# Autodesk Inventor assembly: main room, doors, corridor connected
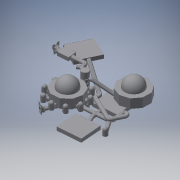
[picture p0: Inventor's stored thumbnail of the model, 180x180]
Saved by Autodesk Inventor 2017 (Build 210142000, 142)
## iProperties
Created: 2018-03-04
Part Number: main room, doors, corridor connected
Document SubType Name: Assembly
Designer: Braxton
Author: Braxton
## Documents named in this file (21)
- E:\School\Game develpment\geoscape\done solid\map (one wall)\main room, doors, corridor connected (one wall).iam
- E:\School\Game develpment\geoscape\done solid\rooms  (one wall)\assembly\main room with double door.iam
- E:\School\Game develpment\geoscape\done solid\doors\end door\9 foot door\end door room (9).ipt
- E:\School\Game develpment\geoscape\done solid\doors\end door\9 foot door\end door assembly (closed) (9).ipt.iam
- E:\School\Game develpment\geoscape\done solid\corridors (one wall done)\corridor (one wall).ipt
- E:\School\Game develpment\geoscape\done solid\corridors (one wall done)\corridor turn (one wall).ipt
- E:\School\Game develpment\geoscape\done solid\corridors (one wall done)\Y corridor  (one wall).ipt
- E:\School\Game develpment\geoscape\done solid\corridors (one wall done)\end cap (one wall).ipt
- E:\School\Game develpment\geoscape\done solid\corridors (one wall done)\curve ramp (one wall).ipt
- E:\School\Game develpment\geoscape\done solid\corridors (one wall done)\ramp top connect  (one wall).ipt
- E:\School\Game develpment\geoscape\done solid\corridors (one wall done)\ramp (one wall).ipt
- E:\School\Game develpment\geoscape\done solid\corridors (one wall done)\ramp bottom connect (one wall).ipt
- E:\School\Game develpment\geoscape\done solid\rooms  (one wall)\assembly\assembly of dome with corridors with all doors.iam
- E:\School\Game develpment\geoscape\done solid\rooms  (one wall)\assembly\dome one terminal.iam
- E:\School\Game develpment\geoscape\done solid\corridors (one wall done)\X corridor  (one wall).ipt
- E:\School\Game develpment\geoscape\done solid\corridors (one wall done)\ramp connect both ends  (one wall).ipt
- E:\School\Game develpment\geoscape\done solid\rooms  (one wall)\room with 15 cubicals (one wall).ipt
- E:\School\Game develpment\geoscape\done solid\doors\end door\9 foot door\end door assembly (9).ipt.iam
- E:\School\Game develpment\geoscape\done solid\rooms  (one wall)\assembly\dome with double door.iam
- end door assembly (closed) (9).ipt
- end door assembly (9).ipt
## Components (70 placed, 18 different names)
1. corridor (one wall):19 — Flush:52, Mate:15, Insert:66, Insert:67
2. corridor (one wall):18 — Flush:51, Flush:52, Insert:65, Insert:66
3. corridor (one wall):17 — Flush:50, Flush:51, Insert:64, Insert:65
4. corridor (one wall):16 — Flush:49, Flush:50, Insert:63, Insert:64
5. corridor (one wall):15 — Flush:48, Flush:49, Insert:62, Insert:63
6. corridor turn (one wall):8 — Mate:14, Flush:48, Insert:61, Insert:62
7. ramp top connect  (one wall):3 — Flush:47, Insert:57, Insert:60, Mate:11
8. ramp (one wall):8 — Flush:46, Flush:47, Insert:56, Insert:57
9. ramp (one wall):7 — Flush:45, Flush:46, Insert:55, Insert:56
10. ramp (one wall):6 — Flush:44, Flush:45, Insert:54, Insert:55
11. ramp (one wall):5 — Flush:43, Flush:44, Insert:53, Insert:54
12. ramp (one wall):4 — Flush:42, Flush:43, Insert:52, Insert:53
13. ramp bottom connect (one wall):3 — Insert:51, Flush:42, Insert:52
14. corridor turn (one wall):7 — Insert:49, Flush:41, Insert:51
15. corridor turn (one wall):6 — Insert:49, Insert:50, Flush:40, Flush:41
16. corridor (one wall):14 — Flush:36, Insert:48, Insert:50, Flush:40
17. corridor (one wall):13 — Flush:36, Flush:37, Insert:47, Insert:48
18. corridor (one wall):12 — Flush:37, Flush:38, Insert:46, Insert:47
19. corridor (one wall):11 — Flush:38, Flush:39, Insert:45, Insert:46
20. corridor (one wall):10 — Flush:39, Insert:44, Insert:45
21. corridor turn (one wall):5 — Flush:34, Insert:42, Insert:44
22. corridor (one wall):9 — Flush:33, Flush:34, Insert:41, Insert:42
23. corridor (one wall):8 — Flush:32, Flush:33, Insert:40, Insert:41
24. corridor turn (one wall):4 — Flush:31, Flush:32, Insert:39, Insert:40
25. corridor turn (one wall):3 — Flush:30, Flush:31, Insert:38, Insert:39
26. ramp top connect  (one wall):2 — Insert:37, Flush:29, Flush:30, Insert:38
27. ramp bottom connect (one wall):2 — Insert:37, Flush:29, Insert:43, Flush:35
28. corridor (one wall):7 — Insert:35, Flush:28, Mate:10
29. corridor (one wall):6 — Insert:34, Insert:35, Flush:27, Flush:28
30. Y corridor  (one wall):2 — Insert:33, Flush:26, Insert:34, Flush:27, Insert:43, Flush:35
31. corridor (one wall):5 — Insert:32, Insert:33, Flush:25, Flush:26
32. ramp connect both ends  (one wall):2 — Insert:30, Flush:24, Insert:58, Mate:12
33. ramp connect both ends  (one wall):1 — Insert:29, Flush:23, Insert:59, Mate:13
34. X corridor  (one wall):1 — Insert:28, Insert:29, Insert:30, Flush:22, Flush:23, Flush:24, Insert:32, Flush:25
35. corridor (one wall):4 — Insert:27, Insert:28, Flush:21, Flush:22
36. corridor (one wall):3 — Insert:26, Insert:27, Flush:20, Flush:21
37. corridor turn (one wall):2 — Insert:26, Insert:31, Mate:9, Flush:20
38. end cap (one wall):3 — Insert:25, Mate:8
39. end cap (one wall):2 — Insert:24, Mate:7
40. ramp bottom connect (one wall):1 — Insert:12, Flush:9, Insert:78, Mate:18
41. ramp (one wall):3 — Insert:11, Flush:8, Insert:12, Flush:9
42. ramp (one wall):2 — Insert:10, Insert:11, Flush:7, Flush:8
43. ramp (one wall):1 — Insert:9, Insert:10, Flush:6, Flush:7
44. ramp top connect  (one wall):1 — Insert:8, Mate:5, Insert:9, Flush:6
45. curve ramp (one wall):1 — Insert:7, Mate:4, Insert:8, Mate:5, Flush:10, Insert:24, Mate:7, Insert:25, Mate:8, Insert:31, Mate:9, Mate:14, Insert:61, Insert:77
46. end cap (one wall):1 — Insert:6, Flush:5
47. Y corridor  (one wall):1 — Insert:5, Flush:4, Insert:6, Flush:5, Insert:7, Mate:4
48. corridor turn (one wall):1 — Insert:4, Flush:3, Insert:5, Flush:4
49. corridor (one wall):2 — Insert:3, Flush:2, Insert:4, Flush:3
50. corridor (one wall):1 — Insert:2, Insert:3, Mate:3, Flush:2
51. room with 15 cubicals (one wall):1 — Insert:58, Mate:12
52. room with 15 cubicals (one wall):2 — Insert:59, Mate:13
53. room with 15 cubicals (one wall):3 — Insert:60, Mate:11
54. assembly of dome with corridors with all doors:1 [sub-assembly] — Flush:10, Flush:11, Flush:12, Flush:13, Flush:14, Flush:15, Flush:16, Flush:17, Flush:18, Flush:19, Insert:68, Insert:69, Insert:70, Insert:71, Insert:72, Insert:73, Insert:74, Insert:75, Insert:76, Insert:77
55. main room with double door:1 [sub-assembly] — Insert:1, Flush:1, Insert:2, Mate:3
56. end door room (9):2 — Mate:15, Insert:67, Mate:16, Mate:17
57. end door assembly (9).ipt:1 [sub-assembly] — Mate:16, Mate:17
58. end door assembly (closed) (9).ipt:1 [sub-assembly] — Mate:1, Mate:2
59. end door room (9):1 — Insert:1, Flush:1, Mate:1, Mate:2
60. dome with double door:1 [sub-assembly] — Insert:78, Mate:18
61. dome one terminal:10 [sub-assembly] — Mate:10
62. dome one terminal:1 [sub-assembly] — Flush:19, Insert:76
63. dome one terminal:2 [sub-assembly] — Flush:18, Insert:75
64. dome one terminal:3 [sub-assembly] — Flush:17, Insert:74
65. dome one terminal:4 [sub-assembly] — Flush:16, Insert:73
66. dome one terminal:5 [sub-assembly] — Flush:15, Insert:72
67. dome one terminal:6 [sub-assembly] — Flush:14, Insert:71
68. dome one terminal:7 [sub-assembly] — Flush:13, Insert:70
69. dome one terminal:8 [sub-assembly] — Flush:12, Insert:69
70. dome one terminal:9 [sub-assembly] — Flush:11, Insert:68
## Relationships (135: Insert 66, Flush 52, Mate 17)
- Insert:1: main room with double door:1 ↔ end door room (9):1
- Flush:1: main room with double door:1 ↔ end door room (9):1
- Mate:1: end door assembly (closed) (9).ipt:1 ↔ end door room (9):1
- Mate:2: end door assembly (closed) (9).ipt:1 ↔ end door room (9):1
- Insert:2: corridor (one wall):1 ↔ main room with double door:1
- Insert:3: corridor (one wall):2 ↔ corridor (one wall):1
- Mate:3: corridor (one wall):1 ↔ main room with double door:1
- Flush:2: corridor (one wall):2 ↔ corridor (one wall):1
- Insert:4: corridor turn (one wall):1 ↔ corridor (one wall):2
- Flush:3: corridor turn (one wall):1 ↔ corridor (one wall):2
- Insert:5: Y corridor  (one wall):1 ↔ corridor turn (one wall):1
- Flush:4: Y corridor  (one wall):1 ↔ corridor turn (one wall):1
- Insert:6: end cap (one wall):1 ↔ Y corridor  (one wall):1
- Flush:5: end cap (one wall):1 ↔ Y corridor  (one wall):1
- Insert:7: curve ramp (one wall):1 ↔ Y corridor  (one wall):1
- Mate:4: curve ramp (one wall):1 ↔ Y corridor  (one wall):1
- Insert:8: ramp top connect  (one wall):1 ↔ curve ramp (one wall):1
- Mate:5: ramp top connect  (one wall):1 ↔ curve ramp (one wall):1
- Insert:9: ramp (one wall):1 ↔ ramp top connect  (one wall):1
- Insert:10: ramp (one wall):2 ↔ ramp (one wall):1
- Insert:11: ramp (one wall):3 ↔ ramp (one wall):2
- Flush:6: ramp (one wall):1 ↔ ramp top connect  (one wall):1
- Flush:7: ramp (one wall):2 ↔ ramp (one wall):1
- Flush:8: ramp (one wall):3 ↔ ramp (one wall):2
- Insert:12: ramp bottom connect (one wall):1 ↔ ramp (one wall):3
- Flush:9: ramp bottom connect (one wall):1 ↔ ramp (one wall):3
- Flush:10: curve ramp (one wall):1 ↔ assembly of dome with corridors with all doors:1
- Flush:11: assembly of dome with corridors with all doors:1 ↔ dome one terminal:9
- Flush:12: assembly of dome with corridors with all doors:1 ↔ dome one terminal:8
- Flush:13: assembly of dome with corridors with all doors:1 ↔ dome one terminal:7
- Flush:14: assembly of dome with corridors with all doors:1 ↔ dome one terminal:6
- Flush:15: assembly of dome with corridors with all doors:1 ↔ dome one terminal:5
- Flush:16: assembly of dome with corridors with all doors:1 ↔ dome one terminal:4
- Flush:17: assembly of dome with corridors with all doors:1 ↔ dome one terminal:3
- Flush:18: assembly of dome with corridors with all doors:1 ↔ dome one terminal:2
- Flush:19: assembly of dome with corridors with all doors:1 ↔ dome one terminal:1
- Insert:24: end cap (one wall):2 ↔ curve ramp (one wall):1
- Mate:7: end cap (one wall):2 ↔ curve ramp (one wall):1
- Insert:25: end cap (one wall):3 ↔ curve ramp (one wall):1
- Mate:8: end cap (one wall):3 ↔ curve ramp (one wall):1
- Insert:26: corridor (one wall):3 ↔ corridor turn (one wall):2
- Insert:27: corridor (one wall):4 ↔ corridor (one wall):3
- Insert:28: X corridor  (one wall):1 ↔ corridor (one wall):4
- Insert:29: ramp connect both ends  (one wall):1 ↔ X corridor  (one wall):1
- Insert:30: ramp connect both ends  (one wall):2 ↔ X corridor  (one wall):1
- Insert:31: corridor turn (one wall):2 ↔ curve ramp (one wall):1
- Mate:9: corridor turn (one wall):2 ↔ curve ramp (one wall):1
- Flush:20: corridor (one wall):3 ↔ corridor turn (one wall):2
- Flush:21: corridor (one wall):4 ↔ corridor (one wall):3
- Flush:22: X corridor  (one wall):1 ↔ corridor (one wall):4
- Flush:23: ramp connect both ends  (one wall):1 ↔ X corridor  (one wall):1
- Flush:24: ramp connect both ends  (one wall):2 ↔ X corridor  (one wall):1
- Insert:32: corridor (one wall):5 ↔ X corridor  (one wall):1
- Insert:33: Y corridor  (one wall):2 ↔ corridor (one wall):5
- Flush:25: corridor (one wall):5 ↔ X corridor  (one wall):1
- Flush:26: Y corridor  (one wall):2 ↔ corridor (one wall):5
- Insert:34: corridor (one wall):6 ↔ Y corridor  (one wall):2
- Insert:35: corridor (one wall):7 ↔ corridor (one wall):6
- Flush:27: corridor (one wall):6 ↔ Y corridor  (one wall):2
- Flush:28: corridor (one wall):7 ↔ corridor (one wall):6
- Mate:10: corridor (one wall):7 ↔ dome one terminal:10
- Insert:37: ramp top connect  (one wall):2 ↔ ramp bottom connect (one wall):2
- Flush:29: ramp top connect  (one wall):2 ↔ ramp bottom connect (one wall):2
- Flush:30: corridor turn (one wall):3 ↔ ramp top connect  (one wall):2
- Flush:31: corridor turn (one wall):4 ↔ corridor turn (one wall):3
- Flush:32: corridor (one wall):8 ↔ corridor turn (one wall):4
- Flush:33: corridor (one wall):9 ↔ corridor (one wall):8
- Flush:34: corridor turn (one wall):5 ↔ corridor (one wall):9
- Insert:38: corridor turn (one wall):3 ↔ ramp top connect  (one wall):2
- Insert:39: corridor turn (one wall):4 ↔ corridor turn (one wall):3
- Insert:40: corridor (one wall):8 ↔ corridor turn (one wall):4
- Insert:41: corridor (one wall):9 ↔ corridor (one wall):8
- Insert:42: corridor turn (one wall):5 ↔ corridor (one wall):9
- Insert:43: ramp bottom connect (one wall):2 ↔ Y corridor  (one wall):2
- Flush:35: ramp bottom connect (one wall):2 ↔ Y corridor  (one wall):2
- Flush:36: corridor (one wall):14 ↔ corridor (one wall):13
- Flush:37: corridor (one wall):13 ↔ corridor (one wall):12
- Flush:38: corridor (one wall):12 ↔ corridor (one wall):11
- Flush:39: corridor (one wall):11 ↔ corridor (one wall):10
- Insert:44: corridor (one wall):10 ↔ corridor turn (one wall):5
- Insert:45: corridor (one wall):11 ↔ corridor (one wall):10
- Insert:46: corridor (one wall):12 ↔ corridor (one wall):11
- Insert:47: corridor (one wall):13 ↔ corridor (one wall):12
- Insert:48: corridor (one wall):14 ↔ corridor (one wall):13
- Insert:49: corridor turn (one wall):7 ↔ corridor turn (one wall):6
- Insert:50: corridor turn (one wall):6 ↔ corridor (one wall):14
- Flush:40: corridor turn (one wall):6 ↔ corridor (one wall):14
- Flush:41: corridor turn (one wall):7 ↔ corridor turn (one wall):6
- Insert:51: ramp bottom connect (one wall):3 ↔ corridor turn (one wall):7
- Flush:42: ramp (one wall):4 ↔ ramp bottom connect (one wall):3
- Flush:43: ramp (one wall):5 ↔ ramp (one wall):4
- Flush:44: ramp (one wall):6 ↔ ramp (one wall):5
- Flush:45: ramp (one wall):7 ↔ ramp (one wall):6
- Flush:46: ramp (one wall):8 ↔ ramp (one wall):7
- Flush:47: ramp top connect  (one wall):3 ↔ ramp (one wall):8
- Insert:52: ramp (one wall):4 ↔ ramp bottom connect (one wall):3
- Insert:53: ramp (one wall):5 ↔ ramp (one wall):4
- Insert:54: ramp (one wall):6 ↔ ramp (one wall):5
- Insert:55: ramp (one wall):7 ↔ ramp (one wall):6
- Insert:56: ramp (one wall):8 ↔ ramp (one wall):7
- Insert:57: ramp top connect  (one wall):3 ↔ ramp (one wall):8
- Insert:58: ramp connect both ends  (one wall):2 ↔ room with 15 cubicals (one wall):1
- Insert:59: ramp connect both ends  (one wall):1 ↔ room with 15 cubicals (one wall):2
- Insert:60: ramp top connect  (one wall):3 ↔ room with 15 cubicals (one wall):3
- Mate:11: ramp top connect  (one wall):3 ↔ room with 15 cubicals (one wall):3
- Mate:12: ramp connect both ends  (one wall):2 ↔ room with 15 cubicals (one wall):1
- Mate:13: ramp connect both ends  (one wall):1 ↔ room with 15 cubicals (one wall):2
- Mate:14: corridor turn (one wall):8 ↔ curve ramp (one wall):1
- Flush:48: corridor (one wall):15 ↔ corridor turn (one wall):8
- Flush:49: corridor (one wall):16 ↔ corridor (one wall):15
- Flush:50: corridor (one wall):17 ↔ corridor (one wall):16
- Flush:51: corridor (one wall):18 ↔ corridor (one wall):17
- Flush:52: corridor (one wall):19 ↔ corridor (one wall):18
- Mate:15: corridor (one wall):19 ↔ end door room (9):2
- Insert:61: corridor turn (one wall):8 ↔ curve ramp (one wall):1
- Insert:62: corridor (one wall):15 ↔ corridor turn (one wall):8
- Insert:63: corridor (one wall):16 ↔ corridor (one wall):15
- Insert:64: corridor (one wall):17 ↔ corridor (one wall):16
- Insert:65: corridor (one wall):18 ↔ corridor (one wall):17
- Insert:66: corridor (one wall):19 ↔ corridor (one wall):18
- Insert:67: corridor (one wall):19 ↔ end door room (9):2
- Mate:16: end door room (9):2 ↔ end door assembly (9).ipt:1
- Mate:17: end door room (9):2 ↔ end door assembly (9).ipt:1
- Insert:68: assembly of dome with corridors with all doors:1 ↔ dome one terminal:9
- Insert:69: assembly of dome with corridors with all doors:1 ↔ dome one terminal:8
- Insert:70: assembly of dome with corridors with all doors:1 ↔ dome one terminal:7
- Insert:71: assembly of dome with corridors with all doors:1 ↔ dome one terminal:6
- Insert:72: assembly of dome with corridors with all doors:1 ↔ dome one terminal:5
- Insert:73: assembly of dome with corridors with all doors:1 ↔ dome one terminal:4
- Insert:74: assembly of dome with corridors with all doors:1 ↔ dome one terminal:3
- Insert:75: assembly of dome with corridors with all doors:1 ↔ dome one terminal:2
- Insert:76: assembly of dome with corridors with all doors:1 ↔ dome one terminal:1
- Insert:77: curve ramp (one wall):1 ↔ assembly of dome with corridors with all doors:1
- Insert:78: ramp bottom connect (one wall):1 ↔ dome with double door:1
- Mate:18: ramp bottom connect (one wall):1 ↔ dome with double door:1
